# Autodesk Inventor assembly: rotator_xw
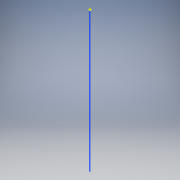
[picture p0: Inventor's stored thumbnail of the model, 180x180]
Saved by Autodesk Inventor 2016 (Build 200138000, 138)
## iProperties
Created: 2015-06-08
Part Number: rotator_xw
Document SubType Name: Assembly
Designer: 121767
Author: 121767
## Documents named in this file (7)
- C:\github\Rotator\Rotator.iam
- C:\github\Rotator\Rotator Frame.ipt
- C:\github\Rotator\Gear platform.ipt
- C:\github\Rotator\Wiring platform.ipt
- C:\github\Rotator\Suspension axle.ipt
- C:\github\Rotator\Suspension bearing.ipt
- C:\github\Rotator\Slotted center beam.ipt
## Components (8 placed, 6 different names)
1. Rotator Frame:1 — Rigid:7, Rigid:8
2. Gear platform:1 — Rigid:1, Rigid:5, Rigid:6
3. Wiring platform:1 — Rigid:1
4. Slotted center beam:1 — Rigid:8
5. Suspension axle:1 — Rotational:3, Rigid:6
6. Suspension axle:2 — Rotational:4, Rigid:5
7. Suspension bearing:1 — Rotational:3
8. Suspension bearing:2 — Rotational:4, Rigid:7
## Relationships (7: WeldJoint 5, RevoluteJoint 2)
- Rigid:1 [WeldJoint]: Gear platform:1 ↔ Wiring platform:1
- Rotational:3 [RevoluteJoint]: Suspension axle:1 ↔ Suspension bearing:1
- Rotational:4 [RevoluteJoint]: Suspension axle:2 ↔ Suspension bearing:2
- Rigid:5 [WeldJoint]: Gear platform:1 ↔ Suspension axle:2
- Rigid:6 [WeldJoint]: Gear platform:1 ↔ Suspension axle:1
- Rigid:7 [WeldJoint]: Rotator Frame:1 ↔ Suspension bearing:2
- Rigid:8 [WeldJoint]: Rotator Frame:1 ↔ Slotted center beam:1
